# Autodesk Inventor assembly: 0012_Bo_truot
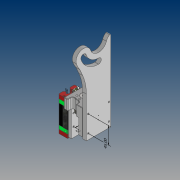
[picture p0: Inventor's stored thumbnail of the model, 180x180]
Saved by Autodesk Inventor 2021 (Build 250183000, 183)
## iProperties
Created: 2024-04-06
Part Number: 0012_Bo_truot
Document SubType Name: Assembly
Designer: Admin
Author: Admin
## Documents named in this file (6)
- C:\Users\Admin\Desktop\DO_AN_TOT_NGHIEP_2024\Mechanical\Design_in_3D\Version_1\0012_Bo_truot.iam
- C:\Users\Admin\Desktop\DO_AN_TOT_NGHIEP_2024\Mechanical\Design_in_3D\Library\hgr-20-1.snapshot.3\HGR20\HGR20.ipt.iam
- C:\Users\Admin\Desktop\DO_AN_TOT_NGHIEP_2024\Mechanical\Design_in_3D\Library\1204-x-430mm-ball-screw-with-bk10-and-bf-bearing-blocks.snapshot.3\1204 BALL NUT.ipt
- C:\Users\Admin\Desktop\DO_AN_TOT_NGHIEP_2024\Mechanical\Design_in_3D\Version_1\20_Khoi_vuong_A.ipt
- C:\Users\Admin\Desktop\DO_AN_TOT_NGHIEP_2024\Mechanical\Design_in_3D\Version_1\16_Khau_hai.ipt
- HGR20.ipt
## Components (4 placed, 4 different names)
1. HGR20.ipt:1 [sub-assembly] — Insert:1, Mate:1
2. 1204 BALL NUT:1 — Flush:1
3. 20_Khoi_vuong_A:1 — Flush:1, Insert:1, Mate:1, Insert:2, Mate:2
4. 16_Khau_hai:1 — Insert:2, Mate:2
## Relationships (5: Insert 2, Mate 2, Flush 1)
- Flush:1: 1204 BALL NUT:1 ↔ 20_Khoi_vuong_A:1
- Insert:1: HGR20.ipt:1 ↔ 20_Khoi_vuong_A:1
- Mate:1: HGR20.ipt:1 ↔ 20_Khoi_vuong_A:1
- Insert:2: 20_Khoi_vuong_A:1 ↔ 16_Khau_hai:1
- Mate:2: 20_Khoi_vuong_A:1 ↔ 16_Khau_hai:1
